# Autodesk Inventor assembly: Pump_V3_Корпус
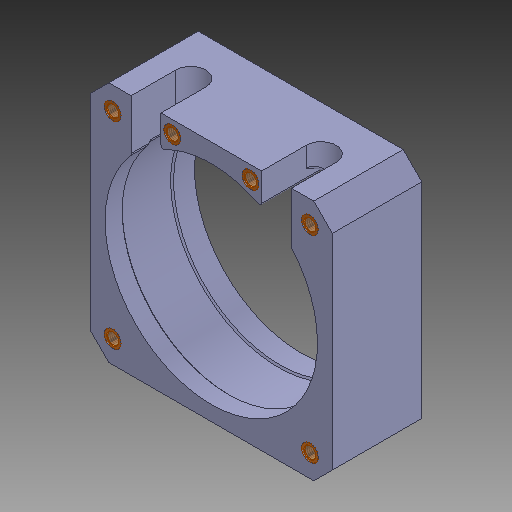
[picture p0: Inventor's stored thumbnail of the model, 512x512]
Saved by Autodesk Inventor 2022 (Build 260153000, 153)
## iProperties
Created: 2025-01-26
Part Number: Pump_V3_Корпус
Document SubType Name: Assembly
Designer: Ivan
Author: Ivan
## Documents named in this file (3)
- E:\4. Прочее\1517\Предпрофессиональная олимпиада\Насос\Itteration_4\Pump_V4_Корпус.iam
- E:\4. Прочее\1517\Предпрофессиональная олимпиада\Насос\Itteration_4\Pump_V4_Корпус.ipt
- E:\4. Прочее\1517\Предпрофессиональная олимпиада\Насос\Itteration_4\Втулка Впаиваемая М3х4.2х5.ipt
## Components (11 placed, 2 different names)
1. Pump_V4_Корпус:1 — Совмещение:5, Совмещение:6, Совмещение:7, Совмещение:8, Заподлицо:5, Заподлицо:6, Заподлицо:7, Заподлицо:8, Совмещение:9, Заподлицо:9, Совмещение:10, Совмещение:11, Совмещение:12, Заподлицо:10, Заподлицо:11, Заподлицо:12, Совмещение:13, Заподлицо:13, Совмещение:14, Заподлицо:14
2. Втулка Впаиваемая М3х4.2х5:5 — Совмещение:7, Заподлицо:8
3. Втулка Впаиваемая М3х4.2х5:6 — Совмещение:6, Заподлицо:7
4. Втулка Впаиваемая М3х4.2х5:7 — Совмещение:5, Заподлицо:5
5. Втулка Впаиваемая М3х4.2х5:8 — Совмещение:8, Заподлицо:6
6. Втулка Впаиваемая М3х4.2х5:9 — Совмещение:9, Заподлицо:9
7. Втулка Впаиваемая М3х4.2х5:10 — Совмещение:12, Заподлицо:10
8. Втулка Впаиваемая М3х4.2х5:11 — Совмещение:10, Заподлицо:12
9. Втулка Впаиваемая М3х4.2х5:12 — Совмещение:11, Заподлицо:11
10. Втулка Впаиваемая М3х4.2х5:13 — Совмещение:13, Заподлицо:13
11. Втулка Впаиваемая М3х4.2х5:14 — Совмещение:14, Заподлицо:14
## Relationships (20: Mate 10, Flush 10)
- Совмещение:5 [Mate]: Pump_V4_Корпус:1 ↔ Втулка Впаиваемая М3х4.2х5:7
- Совмещение:6 [Mate]: Pump_V4_Корпус:1 ↔ Втулка Впаиваемая М3х4.2х5:6
- Совмещение:7 [Mate]: Pump_V4_Корпус:1 ↔ Втулка Впаиваемая М3х4.2х5:5
- Совмещение:8 [Mate]: Pump_V4_Корпус:1 ↔ Втулка Впаиваемая М3х4.2х5:8
- Заподлицо:5 [Flush]: Pump_V4_Корпус:1 ↔ Втулка Впаиваемая М3х4.2х5:7
- Заподлицо:6 [Flush]: Pump_V4_Корпус:1 ↔ Втулка Впаиваемая М3х4.2х5:8
- Заподлицо:7 [Flush]: Pump_V4_Корпус:1 ↔ Втулка Впаиваемая М3х4.2х5:6
- Заподлицо:8 [Flush]: Pump_V4_Корпус:1 ↔ Втулка Впаиваемая М3х4.2х5:5
- Совмещение:9 [Mate]: Pump_V4_Корпус:1 ↔ Втулка Впаиваемая М3х4.2х5:9
- Заподлицо:9 [Flush]: Pump_V4_Корпус:1 ↔ Втулка Впаиваемая М3х4.2х5:9
- Совмещение:10 [Mate]: Pump_V4_Корпус:1 ↔ Втулка Впаиваемая М3х4.2х5:11
- Совмещение:11 [Mate]: Pump_V4_Корпус:1 ↔ Втулка Впаиваемая М3х4.2х5:12
- Совмещение:12 [Mate]: Pump_V4_Корпус:1 ↔ Втулка Впаиваемая М3х4.2х5:10
- Заподлицо:10 [Flush]: Pump_V4_Корпус:1 ↔ Втулка Впаиваемая М3х4.2х5:10
- Заподлицо:11 [Flush]: Pump_V4_Корпус:1 ↔ Втулка Впаиваемая М3х4.2х5:12
- Заподлицо:12 [Flush]: Pump_V4_Корпус:1 ↔ Втулка Впаиваемая М3х4.2х5:11
- Совмещение:13 [Mate]: Pump_V4_Корпус:1 ↔ Втулка Впаиваемая М3х4.2х5:13
- Заподлицо:13 [Flush]: Pump_V4_Корпус:1 ↔ Втулка Впаиваемая М3х4.2х5:13
- Совмещение:14 [Mate]: Pump_V4_Корпус:1 ↔ Втулка Впаиваемая М3х4.2х5:14
- Заподлицо:14 [Flush]: Pump_V4_Корпус:1 ↔ Втулка Впаиваемая М3х4.2х5:14
